# Autodesk Inventor assembly: trussTelescopeTubeAssembly
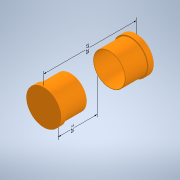
[picture p0: Inventor's stored thumbnail of the model, 180x180]
Saved by Autodesk Inventor 2021.2 (Build 252289000, 289)
## iProperties
Created: 2021-02-11
Part Number: trussTelescopeTubeAssembly
Document SubType Name: Assembly
Designer: robst
Author: robst
## Documents named in this file (3)
- C:\git\CAD-Development\robSteele\ShapeWays\TelescopeProjects\TelescopeMount\trussTelescopeTubeAssembly.iam
- C:\git\CAD-Development\robSteele\ShapeWays\TelescopeProjects\TelescopeMount\trussTelescopeTubeRear.ipt
- C:\git\CAD-Development\robSteele\ShapeWays\TelescopeProjects\TelescopeMount\trussTelescopeTubeFront.ipt
## Components (2 placed, 2 different names)
1. trussTelescopeTubeRear:1 — Mate:1, Mate:2
2. trussTelescopeTubeFront:1 — Mate:1, Mate:2
## Relationships (2: Mate 2)
- Mate:1 (184.15 mm): trussTelescopeTubeRear:1 ↔ trussTelescopeTubeFront:1
- Mate:2: trussTelescopeTubeRear:1 ↔ trussTelescopeTubeFront:1
